# Autodesk Inventor assembly: Color_sensor
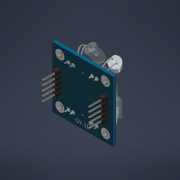
[picture p0: Inventor's stored thumbnail of the model, 180x180]
Saved by Autodesk Inventor 2021 (Build 250183000, 183)
## iProperties
Created: 2016-09-21
Part Number: Color_sensor
Document SubType Name: Assembly
Designer: Ádi
Author: Ádi
## Documents named in this file (9)
- D:\Kien Phan\3D Library\Parts\tcs3200-color-detector\Color_sensor.iam
- D:\Kien Phan\3D Library\Parts\tcs3200-color-detector\Color_sensor_PCB.ipt
- D:\Kien Phan\3D Library\Parts\tcs3200-color-detector\Pin Header 1x5 TH Pitch 2.54mm.ipt
- D:\Kien Phan\3D Library\Parts\tcs3200-color-detector\TCS3200.ipt
- D:\Kien Phan\3D Library\Parts\tcs3200-color-detector\5mm LED.ipt
- D:\Kien Phan\3D Library\Parts\tcs3200-color-detector\5mm LED_MIR.ipt
- D:\Kien Phan\3D Library\Parts\tcs3200-color-detector\5mm LED_MIR1.ipt
- D:\Kien Phan\3D Library\Parts\tcs3200-color-detector\5mm LED_MIR_MIR.ipt
- D:\_Egyéni projektek\univerzális\V0_4_sim\ContentCenter\en-US\GB_T 13806.2-92 A\Screw GB_T 13806.2 A ST1.5 x 4.ipt
## Components (10 placed, 8 different names)
1. Color_sensor_PCB:1 — Mate:1, Mate:2, Mate:3, Mate:4, Mate:5, Mate:6, Mate:7, Mate:8, Mate:9, Mate:10, Insert:1, Insert:2
2. Pin Header 1x5 TH Pitch 2.54mm:1 — Mate:1, Mate:2, Mate:3
3. Pin Header 1x5 TH Pitch 2.54mm:2 — Mate:4, Mate:5, Mate:6
4. TCS3200:1 — Mate:7, Mate:8
5. 5mm LED:1 — Mate:9, Mate:10
6. 5mm LED_MIR:1
7. 5mm LED_MIR1:1
8. 5mm LED_MIR_MIR:1
9. Tapping screw GB/T 13806.2-1992 Type A ST1.5 x 4 - A:1 — Insert:1
10. Tapping screw GB/T 13806.2-1992 Type A ST1.5 x 4 - A:2 — Insert:2
## Relationships (12: Mate 10, Insert 2)
- Mate:1: Color_sensor_PCB:1 ↔ Pin Header 1x5 TH Pitch 2.54mm:1
- Mate:2: Color_sensor_PCB:1 ↔ Pin Header 1x5 TH Pitch 2.54mm:1
- Mate:3: Color_sensor_PCB:1 ↔ Pin Header 1x5 TH Pitch 2.54mm:1
- Mate:4: Color_sensor_PCB:1 ↔ Pin Header 1x5 TH Pitch 2.54mm:2
- Mate:5: Color_sensor_PCB:1 ↔ Pin Header 1x5 TH Pitch 2.54mm:2
- Mate:6: Color_sensor_PCB:1 ↔ Pin Header 1x5 TH Pitch 2.54mm:2
- Mate:7: Color_sensor_PCB:1 ↔ TCS3200:1
- Mate:8: Color_sensor_PCB:1 ↔ TCS3200:1
- Mate:9: Color_sensor_PCB:1 ↔ 5mm LED:1
- Mate:10: Color_sensor_PCB:1 ↔ 5mm LED:1
- Insert:1: Color_sensor_PCB:1 ↔ Tapping screw GB/T 13806.2-1992 Type A ST1.5 x 4 - A:1
- Insert:2: Color_sensor_PCB:1 ↔ Tapping screw GB/T 13806.2-1992 Type A ST1.5 x 4 - A:2
